# Autodesk Inventor assembly: Klapp-Baugruppe
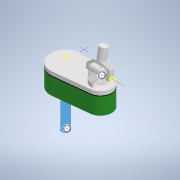
[picture p0: Inventor's stored thumbnail of the model, 180x180]
Saved by Autodesk Inventor 2021 (Build 250183000, 183)
## iProperties
Created: 2021-01-12
Part Number: Klapp-Baugruppe
Document SubType Name: Assembly
Designer: Jaro Machnow
Author: Jaro Machnow
## Documents named in this file (15)
- C:\Users\Jaro Machnow\Documents\Vault\Gruppen\Gruppe 2\Entwurf\Amphibienfahrzeug\Wechsel zwischen Land und Wasser\Wechselmechanik\Klappmechanismus2\Klapp-Baugruppe.iam
- C:\Users\Jaro Machnow\Documents\Vault\Gruppen\Gruppe 2\Entwurf\Amphibienfahrzeug\Wechsel zwischen Land und Wasser\Wechselmechanik\Klappmechanismus\Klapphülle.ipt
- C:\Users\Jaro Machnow\Documents\Vault\Gruppen\Gruppe 2\Entwurf\Amphibienfahrzeug\Wechsel zwischen Land und Wasser\Wechselmechanik\Klappmechanismus\Welle1_zur_Karosserie.ipt
- C:\Users\Jaro Machnow\Documents\Vault\Gruppen\Gruppe 2\Entwurf\Amphibienfahrzeug\Wechsel zwischen Land und Wasser\Wechselmechanik\Klappmechanismus\Kraftübertragung mit Keilriemen.iam
- C:\Users\Jaro Machnow\Documents\Vault\Gruppen\Gruppe 2\Entwurf\Amphibienfahrzeug\Wechsel zwischen Land und Wasser\Wechselmechanik\Klappmechanismus\Welle2_zum_Rad.ipt
- C:\Users\Jaro Machnow\Documents\Vault\Gruppen\Gruppe 2\Entwurf\Amphibienfahrzeug\Wechsel zwischen Land und Wasser\Wechselmechanik\Klappmechanismus\Lager1.iam
- C:\Users\Jaro Machnow\Documents\Vault\Gruppen\Gruppe 2\Entwurf\Amphibienfahrzeug\Wechsel zwischen Land und Wasser\Wechselmechanik\Klappmechanismus\Keilverbindung1.iam
- C:\Users\Jaro Machnow\Documents\Vault\Gruppen\Gruppe 2\Entwurf\Amphibienfahrzeug\Wechsel zwischen Land und Wasser\Wechselmechanik\Klappmechanismus\Keilverbindung2.iam
- C:\Users\Jaro Machnow\Documents\Vault\Gruppen\Gruppe 2\Entwurf\Amphibienfahrzeug\Wechsel zwischen Land und Wasser\Wechselmechanik\Klappmechanismus\Dichtungsgummi.ipt
- C:\Users\Jaro Machnow\Documents\Vault\Gruppen\Gruppe 2\Entwurf\Amphibienfahrzeug\Betrieb an Land\Lenkung\Lenkung_Baugruppe.iam
- C:\Users\Jaro Machnow\Documents\Vault\Gruppen\Gruppe 2\Entwurf\Amphibienfahrzeug\Wechsel zwischen Land und Wasser\Wechselmechanik\Klappmechanismus2\Abdeckung_für_Lenkung.ipt
- C:\Users\Jaro Machnow\Documents\Vault\Gruppen\Gruppe 2\Entwurf\Amphibienfahrzeug\Wechsel zwischen Land und Wasser\Wechselmechanik\Klappmechanismus2\Klapp-Baugruppe\Konstruktions-Assistent\Keilverbindung3.iam
- C:\Users\Jaro Machnow\Documents\Vault\Gruppen\Gruppe 2\Entwurf\Amphibienfahrzeug\Wechsel zwischen Land und Wasser\Wechselmechanik\Klappmechanismus2\Klapp-Baugruppe\Konstruktions-Assistent\Keilverbindung4.iam
- C:\Users\Jaro Machnow\Documents\Vault\Gruppen\Gruppe 2\Entwurf\Amphibienfahrzeug\Betrieb an Land\Lenkung\Lenkteil_zum_Rad.ipt
- C:\Users\Jaro Machnow\Documents\Vault\Gruppen\Gruppe 2\Entwurf\Amphibienfahrzeug\Wechsel zwischen Land und Wasser\Wechselmechanik\Klappmechanismus2\Welle3.ipt
## Components (17 placed, 9 different names)
1. Welle:1 — Passend:1, Fluchtend:2, Passend:5, Fluchtend:6, Passend:10, Passend:11, Passend:12, Winkel:2, Passend:46, Fluchtend:10, Winkel:15, Passend:49
2. Kraftübertragung mit Keilriemen:1 [sub-assembly] — Passend:1, Passend:3, Passend:10, Winkel:2, Winkel:4
3. Welle:2 — Passend:3, Fluchtend:2, Passend:8, Passend:9, Winkel:4, Passend:18, Passend:19, Passend:29, Passend:30, Passend:47, Winkel:14, Passend:48, Passend:52, Fluchtend:11, Winkel:16, Passend:54, Winkel:17
4. Lager:1 [sub-assembly] — Passend:5, Fluchtend:6, Passend:21
5. Lager:2 [sub-assembly] — Passend:8, Passend:9
6. Lager:3 [sub-assembly] — Passend:11, Passend:12
7. Keilverbindung:1 [sub-assembly] — Fluchtend:10, Winkel:15, Passend:49
8. Keilverbindung:2 [sub-assembly] — Passend:47, Winkel:14, Passend:48
9. Lager:4 [sub-assembly] — Passend:18, Passend:19
10. Klapphülle:1 — Passend:21, Passend:22, Passend:23, Passend:24, Passend:29, Passend:30, Passend:33, Passend:34, Passend:46
11. Dichtungsgummi:1 — Passend:22, Passend:23, Passend:24, Passend:32
12. Lenkung_Baugruppe:1 [sub-assembly] — Passend:52, Winkel:17, Passend:56, Winkel:19
13. Abdeckung_für_Lenkung:1 — Passend:32, Passend:33, Passend:34, Passend:55
14. Keilverbindung:3 [sub-assembly] — Fluchtend:11, Winkel:16, Passend:54
15. Lenkteil_zum_Rad:1 — Passend:58, Passend:59, Passend:60
16. Welle:1 — Passend:55, Passend:56, Fluchtend:12, Winkel:18, Passend:57, Winkel:19, Passend:58, Passend:59, Passend:60
17. Keilverbindung:4 [sub-assembly] — Fluchtend:12, Winkel:18, Passend:57
## Relationships (44: Mate 31, Angle 8, Flush 5)
- Passend:1 [Mate]: Welle:1 ↔ Kraftübertragung mit Keilriemen:1
- Passend:3 [Mate]: Kraftübertragung mit Keilriemen:1 ↔ Welle:2
- Fluchtend:2 [Flush]: Welle:1 ↔ Welle:2
- Passend:5 [Mate]: Welle:1 ↔ Lager:1
- Fluchtend:6 [Flush]: Welle:1 ↔ Lager:1
- Passend:8 [Mate]: Welle:2 ↔ Lager:2
- Passend:9 [Mate]: Welle:2 ↔ Lager:2
- Passend:10 [Mate]: Welle:1 ↔ Kraftübertragung mit Keilriemen:1
- Passend:11 [Mate]: Welle:1 ↔ Lager:3
- Passend:12 [Mate]: Welle:1 ↔ Lager:3
- Winkel:2 [Angle] (174.2383 deg): Welle:1 ↔ Kraftübertragung mit Keilriemen:1
- Winkel:4 [Angle] (146.2544 deg): Kraftübertragung mit Keilriemen:1 ↔ Welle:2
- Passend:18 [Mate]: Welle:2 ↔ Lager:4
- Passend:19 [Mate]: Welle:2 ↔ Lager:4
- Passend:21 [Mate]: Lager:1 ↔ Klapphülle:1
- Passend:22 [Mate]: Klapphülle:1 ↔ Dichtungsgummi:1
- Passend:23 [Mate]: Klapphülle:1 ↔ Dichtungsgummi:1
- Passend:24 [Mate]: Klapphülle:1 ↔ Dichtungsgummi:1
- Passend:29 [Mate]: Welle:2 ↔ Klapphülle:1
- Passend:30 [Mate]: Welle:2 ↔ Klapphülle:1
- Passend:32 [Mate]: Dichtungsgummi:1 ↔ Abdeckung_für_Lenkung:1
- Passend:33 [Mate]: Klapphülle:1 ↔ Abdeckung_für_Lenkung:1
- Passend:34 [Mate]: Klapphülle:1 ↔ Abdeckung_für_Lenkung:1
- Passend:46 [Mate] (0.064 mm): Welle:1 ↔ Klapphülle:1
- Passend:47 [Mate] (0.9486 mm): Welle:2 ↔ Keilverbindung:2
- Winkel:14 [Angle] (0 deg): Welle:2 ↔ Keilverbindung:2
- Passend:48 [Mate]: Welle:2 ↔ Keilverbindung:2
- Fluchtend:10 [Flush] (1.0188 mm): Welle:1 ↔ Keilverbindung:1
- Winkel:15 [Angle] (0 deg): Welle:1 ↔ Keilverbindung:1
- Passend:49 [Mate]: Welle:1 ↔ Keilverbindung:1
- Passend:52 [Mate]: Welle:2 ↔ Lenkung_Baugruppe:1
- Fluchtend:11 [Flush]: Welle:2 ↔ Keilverbindung:3
- Winkel:16 [Angle] (0 deg): Welle:2 ↔ Keilverbindung:3
- Passend:54 [Mate]: Welle:2 ↔ Keilverbindung:3
- Winkel:17 [Angle] (154.8976 deg): Welle:2 ↔ Lenkung_Baugruppe:1
- Passend:55 [Mate]: Abdeckung_für_Lenkung:1 ↔ Welle:1
- Passend:56 [Mate]: Lenkung_Baugruppe:1 ↔ Welle:1
- Fluchtend:12 [Flush] (0.371 mm): Welle:1 ↔ Keilverbindung:4
- Winkel:18 [Angle] (0 deg): Welle:1 ↔ Keilverbindung:4
- Passend:57 [Mate]: Welle:1 ↔ Keilverbindung:4
- Winkel:19 [Angle] (173.4856 deg): Lenkung_Baugruppe:1 ↔ Welle:1
- Passend:58 [Mate]: Lenkteil_zum_Rad:1 ↔ Welle:1
- Passend:59 [Mate]: Lenkteil_zum_Rad:1 ↔ Welle:1
- Passend:60 [Mate]: Lenkteil_zum_Rad:1 ↔ Welle:1
